# Autodesk Inventor assembly: Assembly1bhuvan
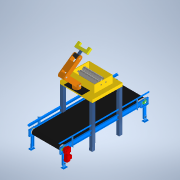
[picture p0: Inventor's stored thumbnail of the model, 180x180]
Saved by Autodesk Inventor 2021 (Build 250183000, 183)
## iProperties
Created: 2021-07-25
Part Number: Assembly1bhuvan
Document SubType Name: Assembly
Designer: aksha
Author: aksha
## Documents named in this file (6)
- C:\akshu\Autodesk\CUP-CRUSHER-NEW\Assembly1bhuvan.iam
- C:\akshu\Autodesk\BHUVAN MECHANICAL-ARM\belt.ipt
- C:\akshu\Autodesk\BHUVAN MECHANICAL-ARM\table.ipt
- C:\akshu\Autodesk\BHUVAN MECHANICAL-ARM\Part7.ipt
- C:\akshu\Autodesk\BHUVAN MECHANICAL-ARM\MECHANICAL ARM (1).iam
- C:\akshu\Autodesk\BHUVAN MECHANICAL-ARM\twister motar 6.ipt
## Components (9 placed, 5 different names)
1. belt:1
2. table:1 — Mate:1, Mate:2, Mate:3, Mate:4, Mate:5, Mate:6, Mate:7, Angle:1, Angle:2
3. MECHANICAL ARM (1):1 [sub-assembly] — Mate:1
4. Part7:1 — Mate:2
5. Part7:2 — Mate:3
6. Part7:3 — Mate:4
7. Part7:4 — Mate:5
8. twister motar 6:1 — Mate:7, Angle:1
9. twister motar 6:2 — Mate:6, Angle:2
## Relationships (9: Mate 7, Angle 2)
- Mate:1: table:1 ↔ MECHANICAL ARM (1):1
- Mate:2: table:1 ↔ Part7:1
- Mate:3: table:1 ↔ Part7:2
- Mate:4: table:1 ↔ Part7:3
- Mate:5: table:1 ↔ Part7:4
- Mate:6: table:1 ↔ twister motar 6:2
- Mate:7: table:1 ↔ twister motar 6:1
- Angle:1 (0 deg): table:1 ↔ twister motar 6:1
- Angle:2 (0 deg): table:1 ↔ twister motar 6:2
